# Autodesk Inventor assembly: assembled
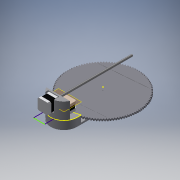
[picture p0: Inventor's stored thumbnail of the model, 180x180]
Saved by Autodesk Inventor 2016 (Build 200138000, 138)
## iProperties
Created: 2016-10-03
Part Number: assembled
Document SubType Name: Assembly
Designer: brent
Author: brent
## Documents named in this file (4)
- C:\Users\brent\OneDrive\classes\desinv22\motorized_drawing_machine\assembled.iam
- C:\Users\brent\OneDrive\classes\desinv22\motorized_drawing_machine\primary.ipt
- C:\Users\brent\OneDrive\classes\desinv22\motorized_drawing_machine\offtheshelf\nema17_40mm_300mml.ipt
- C:\Users\brent\OneDrive\classes\desinv22\motorized_drawing_machine\offtheshelf\nema17_33mm.ipt
## Components (3 placed, 3 different names)
1. primary:1 — Mate:1, Mate:2, Mate:3
2. nema17_40mm_300mml:1 — Mate:2
3. nema17_33mm:1 — Mate:3
## Relationships (3: Mate 3)
- Mate:1: primary:1
- Mate:2: primary:1 ↔ nema17_40mm_300mml:1
- Mate:3: primary:1 ↔ nema17_33mm:1
